# Autodesk Inventor assembly: IntakeSlides5.0
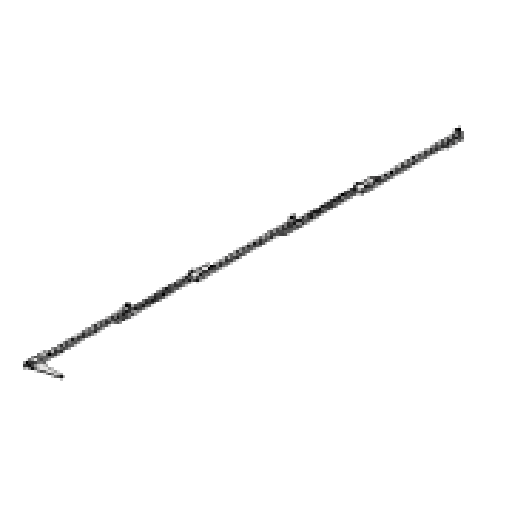
[picture p0: Inventor's stored thumbnail of the model, 512x512]
Saved by Autodesk Inventor 2023 (Build 270158000, 158)
## iProperties
Created: 2022-09-16
Part Number: IntakeSlides5.0
Document SubType Name: Assembly
Designer: deli
Author: deli
## Documents named in this file (9)
- C:\Users\deli\OneDrive - Eastside Preparatory School\FTC\8103-power-play\CAD\IntakeSlides5.0.iam
- C:\Users\deli\OneDrive - Eastside Preparatory School\FTC\8103-power-play\CAD\Carrige.ipt
- C:\Users\deli\OneDrive - Eastside Preparatory School\FTC\8103-power-play\CAD\FTC-parts\Mcmaster Carr\91294A126_Black-Oxide Alloy Steel Hex Drive Flat Head Screw.ipt
- C:\Users\deli\OneDrive - Eastside Preparatory School\FTC\8103-power-play\CAD\mgn9 350mm.ipt
- C:\Users\deli\OneDrive - Eastside Preparatory School\FTC\8103-power-play\CAD\Connector Plate350mm.ipt
- C:\Users\deli\OneDrive - Eastside Preparatory School\FTC\8103-power-play\CAD\mgn9SlideBearingHolder.ipt
- C:\Users\deli\OneDrive - Eastside Preparatory School\FTC\8103-power-play\CAD\Slides Bearings.iam
- C:\Users\deli\OneDrive - Eastside Preparatory School\FTC\8103-power-play\CAD\FTC-parts\M3\hex_socket_button_head_M3x14.ipt
- C:\Users\deli\OneDrive - Eastside Preparatory School\FTC\8103-power-play\CAD\intakeSlidesWheelHolder.ipt
## Components (62 placed, 8 different names)
1. Carrige:3
2. Carrige:4 — Flush:21, Mate:29, Mate:30, Mate:31
3. 91294A126_Black-Oxide Alloy Steel Hex Drive Flat Head Screw:9 — Mate:36, Flush:25
4. 91294A126_Black-Oxide Alloy Steel Hex Drive Flat Head Screw:10 — Mate:34, Flush:28
5. 91294A126_Black-Oxide Alloy Steel Hex Drive Flat Head Screw:11 — Mate:38, Flush:23
6. 91294A126_Black-Oxide Alloy Steel Hex Drive Flat Head Screw:12 — Mate:39, Flush:24
7. 91294A126_Black-Oxide Alloy Steel Hex Drive Flat Head Screw:13 — Mate:32, Flush:29
8. 91294A126_Black-Oxide Alloy Steel Hex Drive Flat Head Screw:14 — Mate:35, Flush:27
9. 91294A126_Black-Oxide Alloy Steel Hex Drive Flat Head Screw:15 — Mate:33, Flush:26
10. 91294A126_Black-Oxide Alloy Steel Hex Drive Flat Head Screw:16 — Mate:37, Flush:22
11. mgn9 350mm:2 — Flush:21, Mate:93, Mate:94, Mate:98
12. Connector Plate350mm:1 — Mate:29, Mate:30, Mate:31, Mate:32, Mate:33, Mate:34, Mate:35, Mate:36, Mate:37, Mate:38, Mate:39, Flush:22, Flush:23, Flush:24, Flush:25, Flush:26, Flush:27, Flush:28, Flush:29, Mate:41, Mate:42, Mate:43, Mate:106, Mate:107, Angle:1, Mate:112, Mate:118, Angle:6
13. Carrige:5 — Mate:41, Mate:42
14. Carrige:6 — Mate:43, Mate:44, Mate:45, Flush:32
15. mgn9 350mm:3 — Mate:44, Mate:45, Flush:32, Mate:46, Mate:47, Mate:48, Mate:49, Mate:50, Mate:51
16. mgn9SlideBearingHolder:1 — Mate:46, Mate:47, Mate:48, Mate:80, Mate:115, Mate:120, Angle:9
17. mgn9SlideBearingHolder:2 — Mate:49, Mate:50, Mate:51, Mate:78, Mate:79, Mate:101, Mate:110, Angle:4
18. Carrige:7
19. Carrige:8
20. 91294A126_Black-Oxide Alloy Steel Hex Drive Flat Head Screw:17
21. 91294A126_Black-Oxide Alloy Steel Hex Drive Flat Head Screw:18
22. 91294A126_Black-Oxide Alloy Steel Hex Drive Flat Head Screw:19
23. 91294A126_Black-Oxide Alloy Steel Hex Drive Flat Head Screw:20
24. 91294A126_Black-Oxide Alloy Steel Hex Drive Flat Head Screw:21
25. 91294A126_Black-Oxide Alloy Steel Hex Drive Flat Head Screw:22
26. 91294A126_Black-Oxide Alloy Steel Hex Drive Flat Head Screw:23
27. 91294A126_Black-Oxide Alloy Steel Hex Drive Flat Head Screw:24
28. mgn9 350mm:4 — Mate:78, Mate:79, Mate:80
29. Connector Plate350mm:2 — Mate:105, Mate:108, Angle:2, Mate:113, Mate:117, Angle:7
30. Carrige:9
31. Carrige:10
32. mgn9 350mm:5 — Mate:142, Mate:143, Mate:144
33. mgn9SlideBearingHolder:3 — Mate:84, Mate:85, Mate:86, Mate:114, Mate:119, Angle:10
34. Carrige:11
35. Carrige:12
36. mgn9 350mm:6 — Mate:84, Mate:85, Mate:86
37. mgn9SlideBearingHolder:5 — Mate:93, Mate:99, Mate:109, Angle:3
38. mgn9SlideBearingHolder:6 — Mate:95, Mate:96, Mate:97, Mate:98, Mate:116, Mate:121, Angle:8
39. Carrige:13
40. Carrige:14
41. mgn9 350mm:7 — Mate:94, Mate:95, Mate:96, Mate:97
42. Slides Bearings:1 [sub-assembly] — Mate:125, Mate:129, Mate:145, Angle:11
43. Slides Bearings:2 [sub-assembly] — Mate:99, Mate:109, Angle:3, Mate:123, Mate:131
44. Slides Bearings:3 [sub-assembly] — Mate:106, Mate:107, Angle:1, Mate:122, Mate:128
45. Slides Bearings:4 [sub-assembly] — Mate:112, Mate:118, Angle:6, Mate:136, Mate:137
46. Slides Bearings:5 [sub-assembly] — Mate:114, Mate:119, Angle:10, Mate:134, Mate:141
47. Slides Bearings:6 [sub-assembly] — Mate:116, Mate:121, Angle:8, Mate:132, Mate:139
48. Slides Bearings:7 [sub-assembly] — Mate:115, Mate:120, Angle:9, Mate:133, Mate:140
49. Slides Bearings:8 [sub-assembly] — Mate:113, Mate:117, Angle:7, Mate:135, Mate:138
50. Slides Bearings:9 [sub-assembly] — Mate:105, Mate:108, Angle:2, Mate:126, Mate:127
51. Slides Bearings:10 [sub-assembly] — Mate:101, Mate:110, Angle:4, Mate:124, Mate:130
52. hex_socket_button_head_M3x14:1 — Mate:124, Mate:130
53. hex_socket_button_head_M3x14:2 — Mate:122, Mate:128
54. hex_socket_button_head_M3x14:3 — Mate:123, Mate:131
55. hex_socket_button_head_M3x14:4 — Mate:126, Mate:127
56. hex_socket_button_head_M3x14:5 — Mate:136, Mate:137
57. hex_socket_button_head_M3x14:6 — Mate:125, Mate:129, Mate:146
58. hex_socket_button_head_M3x14:7 — Mate:135, Mate:138
59. hex_socket_button_head_M3x14:8 — Mate:134, Mate:141
60. hex_socket_button_head_M3x14:9 — Mate:133, Mate:140
61. hex_socket_button_head_M3x14:10 — Mate:132, Mate:139
62. intakeSlidesWheelHolder:1 — Mate:142, Mate:143, Mate:144, Mate:145, Mate:146, Angle:11
## Relationships (157: Mate 113, Flush 34, Angle 10)
- [Flush]: Carrige:3 ↔ Carrige:4
- [Flush]: Carrige:3 ↔ Carrige:4
- [Mate]: Carrige:3 ↔ Carrige:4
- [Mate]: Carrige:4 ↔ mgn9 350mm:2
- [Mate]: Carrige:4 ↔ mgn9 350mm:2
- Flush:21 (292.2 mm): Carrige:4 ↔ mgn9 350mm:2
- Mate:29: Carrige:4 ↔ Connector Plate350mm:1
- Mate:30: Carrige:4 ↔ Connector Plate350mm:1
- Mate:31: Carrige:4 ↔ Connector Plate350mm:1
- Mate:32: 91294A126_Black-Oxide Alloy Steel Hex Drive Flat Head Screw:13 ↔ Connector Plate350mm:1
- Mate:33: 91294A126_Black-Oxide Alloy Steel Hex Drive Flat Head Screw:15 ↔ Connector Plate350mm:1
- Mate:34: 91294A126_Black-Oxide Alloy Steel Hex Drive Flat Head Screw:10 ↔ Connector Plate350mm:1
- Mate:35: 91294A126_Black-Oxide Alloy Steel Hex Drive Flat Head Screw:14 ↔ Connector Plate350mm:1
- Mate:36: 91294A126_Black-Oxide Alloy Steel Hex Drive Flat Head Screw:9 ↔ Connector Plate350mm:1
- Mate:37: 91294A126_Black-Oxide Alloy Steel Hex Drive Flat Head Screw:16 ↔ Connector Plate350mm:1
- Mate:38: 91294A126_Black-Oxide Alloy Steel Hex Drive Flat Head Screw:11 ↔ Connector Plate350mm:1
- Mate:39: 91294A126_Black-Oxide Alloy Steel Hex Drive Flat Head Screw:12 ↔ Connector Plate350mm:1
- Flush:22: 91294A126_Black-Oxide Alloy Steel Hex Drive Flat Head Screw:16 ↔ Connector Plate350mm:1
- Flush:23: 91294A126_Black-Oxide Alloy Steel Hex Drive Flat Head Screw:11 ↔ Connector Plate350mm:1
- Flush:24: 91294A126_Black-Oxide Alloy Steel Hex Drive Flat Head Screw:12 ↔ Connector Plate350mm:1
- Flush:25: 91294A126_Black-Oxide Alloy Steel Hex Drive Flat Head Screw:9 ↔ Connector Plate350mm:1
- Flush:26: 91294A126_Black-Oxide Alloy Steel Hex Drive Flat Head Screw:15 ↔ Connector Plate350mm:1
- Flush:27: 91294A126_Black-Oxide Alloy Steel Hex Drive Flat Head Screw:14 ↔ Connector Plate350mm:1
- Flush:28: 91294A126_Black-Oxide Alloy Steel Hex Drive Flat Head Screw:10 ↔ Connector Plate350mm:1
- Flush:29: 91294A126_Black-Oxide Alloy Steel Hex Drive Flat Head Screw:13 ↔ Connector Plate350mm:1
- [Flush]: Carrige:5 ↔ Carrige:6
- [Flush]: Carrige:5 ↔ Carrige:6
- [Mate]: Carrige:5 ↔ Carrige:6
- Mate:41: Connector Plate350mm:1 ↔ Carrige:5
- Mate:42: Connector Plate350mm:1 ↔ Carrige:5
- Mate:43: Connector Plate350mm:1 ↔ Carrige:6
- Mate:44: Carrige:6 ↔ mgn9 350mm:3
- Mate:45: Carrige:6 ↔ mgn9 350mm:3
- Flush:32 (292.2 mm): Carrige:6 ↔ mgn9 350mm:3
- Mate:46: mgn9 350mm:3 ↔ mgn9SlideBearingHolder:1
- Mate:47: mgn9 350mm:3 ↔ mgn9SlideBearingHolder:1
- Mate:48: mgn9 350mm:3 ↔ mgn9SlideBearingHolder:1
- Mate:49: mgn9 350mm:3 ↔ mgn9SlideBearingHolder:2
- Mate:50: mgn9 350mm:3 ↔ mgn9SlideBearingHolder:2
- Mate:51: mgn9 350mm:3 ↔ mgn9SlideBearingHolder:2
- [Flush]: Carrige:7 ↔ Carrige:8
- [Flush]: Carrige:7 ↔ Carrige:8
- [Mate]: Carrige:7 ↔ Carrige:8
- [Mate]: Carrige:8 ↔ mgn9 350mm:4
- [Mate]: Carrige:8 ↔ mgn9 350mm:4
- [Flush] (292.2 mm): Carrige:8 ↔ mgn9 350mm:4
- [Mate]: Carrige:8 ↔ Connector Plate350mm:2
- [Mate]: Carrige:8 ↔ Connector Plate350mm:2
- [Mate]: Carrige:8 ↔ Connector Plate350mm:2
- [Mate]: 91294A126_Black-Oxide Alloy Steel Hex Drive Flat Head Screw:21 ↔ Connector Plate350mm:2
- [Mate]: 91294A126_Black-Oxide Alloy Steel Hex Drive Flat Head Screw:23 ↔ Connector Plate350mm:2
- [Mate]: 91294A126_Black-Oxide Alloy Steel Hex Drive Flat Head Screw:18 ↔ Connector Plate350mm:2
- [Mate]: 91294A126_Black-Oxide Alloy Steel Hex Drive Flat Head Screw:22 ↔ Connector Plate350mm:2
- [Mate]: 91294A126_Black-Oxide Alloy Steel Hex Drive Flat Head Screw:17 ↔ Connector Plate350mm:2
- [Mate]: 91294A126_Black-Oxide Alloy Steel Hex Drive Flat Head Screw:24 ↔ Connector Plate350mm:2
- [Mate]: 91294A126_Black-Oxide Alloy Steel Hex Drive Flat Head Screw:19 ↔ Connector Plate350mm:2
- [Mate]: 91294A126_Black-Oxide Alloy Steel Hex Drive Flat Head Screw:20 ↔ Connector Plate350mm:2
- [Flush]: 91294A126_Black-Oxide Alloy Steel Hex Drive Flat Head Screw:24 ↔ Connector Plate350mm:2
- [Flush]: 91294A126_Black-Oxide Alloy Steel Hex Drive Flat Head Screw:19 ↔ Connector Plate350mm:2
- [Flush]: 91294A126_Black-Oxide Alloy Steel Hex Drive Flat Head Screw:20 ↔ Connector Plate350mm:2
- [Flush]: 91294A126_Black-Oxide Alloy Steel Hex Drive Flat Head Screw:17 ↔ Connector Plate350mm:2
- [Flush]: 91294A126_Black-Oxide Alloy Steel Hex Drive Flat Head Screw:23 ↔ Connector Plate350mm:2
- [Flush]: 91294A126_Black-Oxide Alloy Steel Hex Drive Flat Head Screw:22 ↔ Connector Plate350mm:2
- [Flush]: 91294A126_Black-Oxide Alloy Steel Hex Drive Flat Head Screw:18 ↔ Connector Plate350mm:2
- [Flush]: 91294A126_Black-Oxide Alloy Steel Hex Drive Flat Head Screw:21 ↔ Connector Plate350mm:2
- [Flush]: Carrige:9 ↔ Carrige:10
- [Flush]: Carrige:9 ↔ Carrige:10
- [Mate]: Carrige:9 ↔ Carrige:10
- [Mate]: Connector Plate350mm:2 ↔ Carrige:9
- [Mate]: Connector Plate350mm:2 ↔ Carrige:9
- [Mate]: Connector Plate350mm:2 ↔ Carrige:10
- [Mate]: Carrige:10 ↔ mgn9 350mm:5
- [Mate]: Carrige:10 ↔ mgn9 350mm:5
- [Flush] (292.2 mm): Carrige:10 ↔ mgn9 350mm:5
- [Mate]: mgn9 350mm:5 ↔ mgn9SlideBearingHolder:3
- [Mate]: mgn9 350mm:5 ↔ mgn9SlideBearingHolder:3
- [Mate]: mgn9 350mm:5 ↔ mgn9SlideBearingHolder:3
- Mate:78: mgn9SlideBearingHolder:2 ↔ mgn9 350mm:4
- Mate:79: mgn9SlideBearingHolder:2 ↔ mgn9 350mm:4
- Mate:80: mgn9SlideBearingHolder:1 ↔ mgn9 350mm:4
- [Flush]: Carrige:11 ↔ Carrige:12
- [Flush]: Carrige:11 ↔ Carrige:12
- [Mate]: Carrige:11 ↔ Carrige:12
- [Mate]: Carrige:12 ↔ mgn9 350mm:6
- [Mate]: Carrige:12 ↔ mgn9 350mm:6
- [Flush] (292.2 mm): Carrige:12 ↔ mgn9 350mm:6
- Mate:84: mgn9SlideBearingHolder:3 ↔ mgn9 350mm:6
- Mate:85: mgn9SlideBearingHolder:3 ↔ mgn9 350mm:6
- Mate:86: mgn9SlideBearingHolder:3 ↔ mgn9 350mm:6
- [Flush]: Carrige:13 ↔ Carrige:14
- [Flush]: Carrige:13 ↔ Carrige:14
- [Mate]: Carrige:13 ↔ Carrige:14
- [Mate]: Carrige:14 ↔ mgn9 350mm:7
- [Mate]: Carrige:14 ↔ mgn9 350mm:7
- [Flush] (292.2 mm): Carrige:14 ↔ mgn9 350mm:7
- [Mate]: mgn9SlideBearingHolder:5 ↔ mgn9 350mm:7
- [Mate]: mgn9SlideBearingHolder:5 ↔ mgn9 350mm:7
- [Mate]: mgn9SlideBearingHolder:5 ↔ mgn9 350mm:7
- Mate:93: mgn9 350mm:2 ↔ mgn9SlideBearingHolder:5
- Mate:94: mgn9 350mm:2 ↔ mgn9 350mm:7
- Mate:95: mgn9SlideBearingHolder:6 ↔ mgn9 350mm:7
- Mate:96: mgn9SlideBearingHolder:6 ↔ mgn9 350mm:7
- Mate:97: mgn9SlideBearingHolder:6 ↔ mgn9 350mm:7
- Mate:98: mgn9 350mm:2 ↔ mgn9SlideBearingHolder:6
- Mate:99: mgn9SlideBearingHolder:5 ↔ Slides Bearings:2
- Mate:101: mgn9SlideBearingHolder:2 ↔ Slides Bearings:10
- Mate:105: Connector Plate350mm:2 ↔ Slides Bearings:9
- Mate:106: Connector Plate350mm:1 ↔ Slides Bearings:3
- Mate:107: Connector Plate350mm:1 ↔ Slides Bearings:3
- Mate:108: Connector Plate350mm:2 ↔ Slides Bearings:9
- Angle:1 (0 deg): Connector Plate350mm:1 ↔ Slides Bearings:3
- Angle:2 (0 deg): Connector Plate350mm:2 ↔ Slides Bearings:9
- Mate:109: mgn9SlideBearingHolder:5 ↔ Slides Bearings:2
- Mate:110: mgn9SlideBearingHolder:2 ↔ Slides Bearings:10
- Mate:112: Connector Plate350mm:1 ↔ Slides Bearings:4
- Mate:113: Connector Plate350mm:2 ↔ Slides Bearings:8
- Mate:114: mgn9SlideBearingHolder:3 ↔ Slides Bearings:5
- Mate:115: mgn9SlideBearingHolder:1 ↔ Slides Bearings:7
- Mate:116: mgn9SlideBearingHolder:6 ↔ Slides Bearings:6
- Mate:117: Connector Plate350mm:2 ↔ Slides Bearings:8
- Mate:118: Connector Plate350mm:1 ↔ Slides Bearings:4
- Mate:119: mgn9SlideBearingHolder:3 ↔ Slides Bearings:5
- Mate:120: mgn9SlideBearingHolder:1 ↔ Slides Bearings:7
- Mate:121: mgn9SlideBearingHolder:6 ↔ Slides Bearings:6
- Angle:3 (0 deg): mgn9SlideBearingHolder:5 ↔ Slides Bearings:2
- Angle:4 (0 deg): mgn9SlideBearingHolder:2 ↔ Slides Bearings:10
- Angle:6 (0 deg): Connector Plate350mm:1 ↔ Slides Bearings:4
- Angle:7 (0 deg): Connector Plate350mm:2 ↔ Slides Bearings:8
- Angle:8 (0 deg): mgn9SlideBearingHolder:6 ↔ Slides Bearings:6
- Angle:9 (0 deg): mgn9SlideBearingHolder:1 ↔ Slides Bearings:7
- Angle:10 (0 deg): mgn9SlideBearingHolder:3 ↔ Slides Bearings:5
- Mate:122: Slides Bearings:3 ↔ hex_socket_button_head_M3x14:2
- Mate:123: Slides Bearings:2 ↔ hex_socket_button_head_M3x14:3
- Mate:124: Slides Bearings:10 ↔ hex_socket_button_head_M3x14:1
- Mate:125: Slides Bearings:1 ↔ hex_socket_button_head_M3x14:6
- Mate:126: Slides Bearings:9 ↔ hex_socket_button_head_M3x14:4
- Mate:127: Slides Bearings:9 ↔ hex_socket_button_head_M3x14:4
- Mate:128: Slides Bearings:3 ↔ hex_socket_button_head_M3x14:2
- Mate:129: Slides Bearings:1 ↔ hex_socket_button_head_M3x14:6
- Mate:130: Slides Bearings:10 ↔ hex_socket_button_head_M3x14:1
- Mate:131: Slides Bearings:2 ↔ hex_socket_button_head_M3x14:3
- Mate:132: Slides Bearings:6 ↔ hex_socket_button_head_M3x14:10
- Mate:133: Slides Bearings:7 ↔ hex_socket_button_head_M3x14:9
- Mate:134: Slides Bearings:5 ↔ hex_socket_button_head_M3x14:8
- Mate:135: Slides Bearings:8 ↔ hex_socket_button_head_M3x14:7
- Mate:136: Slides Bearings:4 ↔ hex_socket_button_head_M3x14:5
- Mate:137: Slides Bearings:4 ↔ hex_socket_button_head_M3x14:5
- Mate:138: Slides Bearings:8 ↔ hex_socket_button_head_M3x14:7
- Mate:139: Slides Bearings:6 ↔ hex_socket_button_head_M3x14:10
- Mate:140: Slides Bearings:7 ↔ hex_socket_button_head_M3x14:9
- Mate:141: Slides Bearings:5 ↔ hex_socket_button_head_M3x14:8
- Mate:142: mgn9 350mm:5 ↔ intakeSlidesWheelHolder:1
- Mate:143: mgn9 350mm:5 ↔ intakeSlidesWheelHolder:1
- Mate:144: mgn9 350mm:5 ↔ intakeSlidesWheelHolder:1
- Mate:145: Slides Bearings:1 ↔ intakeSlidesWheelHolder:1
- Mate:146: hex_socket_button_head_M3x14:6 ↔ intakeSlidesWheelHolder:1
- Angle:11 (0 deg): Slides Bearings:1 ↔ intakeSlidesWheelHolder:1
## Named parameters: stroke = 292.2 mm, d170_d117 = 0 mm, d171_d118 = 0 mm, d172_d119 = 0 mm, d192_d148 = 0 mm, d542_d170_d117 = 0 mm, d543_d171_d118 = 0 mm, d544_d172_d119 = 0 mm, d559_d523 = 0 mm, d560_d524 = 0 mm, d561_d525 = 0 mm, d562_d526 = 0 mm, d563_d527 = 0 mm, d564_d528 = 0 mm, d565_d149 = 0 mm, d566_d170_d117 = 0 mm, d567_d171_d118 = 0 mm, d568_d172_d119 = 0 mm, d569_d192_d148 = 0 mm, d570_d330 = 292.2 mm, d572_d529 = 0 mm, d573_d530 = 0 mm, d574_d531 = 0 mm, d575_d532 = 0 mm, d576_d533 = 0 mm, d577_d534 = 0 mm, d578_d535 = 0 mm, d579_d536 = 0 mm, d580_d537 = 0 mm, d581_d538 = 0 mm, d582_d539 = 0 mm, d583_d540 = 0 mm, d584_d541 = 0 mm, d585_d542_d170_d117 = 0 mm, d586_d543_d171_d118 = 0 mm, d587_d544_d172_d119 = 0 mm, d588_d545 = 0 mm, d589_d546 = 0 mm, d590_d547 = 0 mm, d591_d548 = 0 mm, d592_d549 = 0 mm, d593_d550 = 292.2 mm, d594_d551 = 0 mm, d595_d552 = 0 mm, d596_d553 = 0 mm, d603_d565_d149 = 0 mm, d604_d566_d170_d117 = 0 mm, d605_d567_d171_d118 = 0 mm, d606_d568_d172_d119 = 0 mm, d607_d569_d192_d148 = 0 mm, d608_d570_d330 = 292.2 mm, d613_d603_d565_d149 = 0 mm, d614_d604_d566_d170_d117 = 0 mm, d615_d605_d567_d171_d118 = 0 mm, d616_d606_d568_d172_d119 = 0 mm, d617_d607_d569_d192_d148 = 0 mm, d618_d608_d570_d330 = 292.2 mm, d620_d610 = 0 mm, d621_d611 = 0 mm, d622_d612 = 0 mm
